# Autodesk Inventor assembly: MP1-1001_CAM3
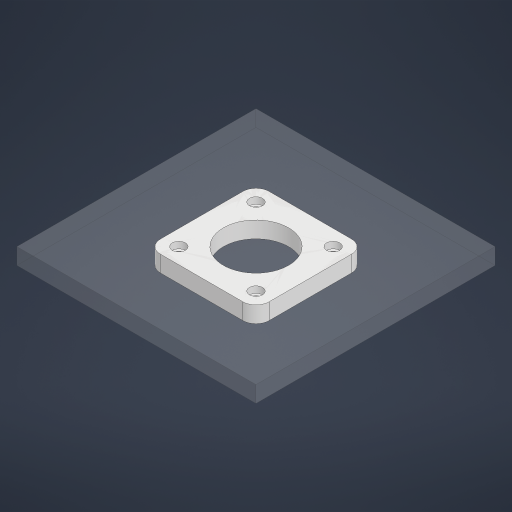
[picture p0: Inventor's stored thumbnail of the model, 512x512]
Saved by Autodesk Inventor 2024.1 (Build 281209000, 209)
## iProperties
Created: 2024-04-04
Part Number: MP1-1001_CAM3
Document SubType Name: Assembly
Designer: fablabadmin
Author: fablabadmin
## Documents named in this file (3)
- C:\Users\fablabadmin\Documents\_Benjamin_S\_3dCAD\HHVerkstad\MountPlate\_CAM\MP1-1001_CAM3.iam
- C:\Users\fablabadmin\Documents\_Benjamin_S\_3dCAD\HHVerkstad\MountPlate\MP1-1001.ipt
- C:\Users\fablabadmin\Documents\_Benjamin_S\_3dCAD\HHVerkstad\MountPlate\_CAM\SquareStock-200-200-15.ipt
## Components (2 placed, 2 different names)
1. MP1-1001:1 — Flush:1
2. SquareStock-200-200-15:1 — Flush:1, Flush:2, Flush:3
## Relationships (3: Flush 3)
- Flush:1: MP1-1001:1 ↔ SquareStock-200-200-15:1
- Flush:2: SquareStock-200-200-15:1
- Flush:3: SquareStock-200-200-15:1
